# Autodesk Inventor assembly: Ensamble
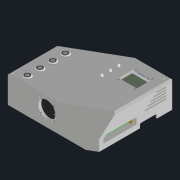
[picture p0: Inventor's stored thumbnail of the model, 180x180]
Saved by Autodesk Inventor 2022 (Build 260153000, 153)
## iProperties
Created: 2022-01-04
Part Number: Ensamble
Document SubType Name: Assembly
Designer: Andres
Author: Andres
## Documents named in this file (22)
- D:\Documentos\Proyectos Personales\SistemaSeguridad\cad\Ensamble.iam
- D:\Documentos\Proyectos Personales\SistemaSeguridad\cad\base.ipt
- D:\Documentos\Proyectos Personales\SistemaSeguridad\cad\mainboard.ipt
- D:\Documentos\Proyectos Personales\SistemaSeguridad\cad\Ardi_UNO.ipt
- D:\Documentos\Proyectos Personales\SistemaSeguridad\cad\4_Relay_module_Simplify_1.ipt
- D:\Documentos\Proyectos Personales\SistemaSeguridad\cad\nokia-5110-lcd-graphic-84x48-pixel-arduiono-compatible-blue-board-1.snapshot.2\Nokia LCD.ipt
- D:\Documentos\Proyectos Personales\SistemaSeguridad\cad\AC-DC transformer.ipt
- D:\Documentos\Proyectos Personales\SistemaSeguridad\cad\Cubierta.ipt
- D:\Documentos\Inventor\Content Center Files\R2022\en-US\ISO 4762(2)\ISO 4762 - M3 x 30ISO.ipt
- D:\Documentos\Inventor\Content Center Files\R2022\en-US\ISO 4032(2)\ISO 4032 - M3 - ISO.ipt
- D:\Documentos\Inventor\Content Center Files\R2022\en-US\ISO 4762(2)\ISO 4762 - M3 x 8ISO.ipt
- D:\Documentos\Proyectos Personales\SistemaSeguridad\cad\led-push-button-1.snapshot.1\LED-BUTTON.ipt
- D:\Documentos\Proyectos Personales\SistemaSeguridad\cad\speaker.ipt
- D:\Documentos\Proyectos Personales\SistemaSeguridad\cad\40x40x10mm-brushless-axial-fan-1.snapshot.2\model.ipt
- fan.ipt
- D:\Documentos\Proyectos Personales\SistemaSeguridad\cad\led-5mm-1.snapshot.6\LED 5mm.ipt
- D:\Documentos\Proyectos Personales\SistemaSeguridad\cad\spacer-m3-l5-l70-1.snapshot.2\Spacer Bolts_m3_bn_L6.ipt
- D:\Documentos\Inventor\Content Center Files\R2022\en-US\ISO 7045  Z\ISO 7045 - M2.5 x 4_ - 4.8 - Z - ISO.ipt
- D:\Documentos\Inventor\Content Center Files\R2022\en-US\ISO 7045  Z\ISO 7045 - M3 x 5_ - 4.8 - Z - ISO.ipt
- D:\Documentos\Inventor\Content Center Files\R2022\en-US\ISO 7045  Z\ISO 7045 - M2.5 x 5_ - 4.8 - Z - ISO.ipt
- D:\Documentos\Inventor\Content Center Files\R2022\en-US\ISO 4762(2)\ISO 4762 - M3 x 12ISO.ipt
- D:\Documentos\Inventor\Content Center Files\R2022\en-US\ISO 4762(2)\ISO 4762 - M3 x 16ISO.ipt
## Components (79 placed, 20 different names)
1. base:1 — Mate:1, Mate:2, Mate:3, Flush:5, Flush:6, Flush:7, Flush:8, Flush:9, Mate:5, Flush:10, Mate:13, Mate:15, Mate:41, Mate:42, Angle:1, Mate:72, Mate:73, Mate:74, Mate:75, Mate:76, Mate:77, Mate:78, Mate:79, Mate:80, Mate:81, Mate:82, Mate:83, Mate:84, Mate:85, Mate:86, Mate:87, Mate:88, Mate:89, Mate:90, Mate:91, Mate:92, Mate:93, Mate:94, Mate:95, Mate:104
2. mainboard:1 — Mate:1, Flush:6, Mate:4, Mate:40, Flush:11, Mate:96, Mate:97, Mate:98, Mate:99, Mate:100, Mate:101, Mate:102, Mate:103, Mate:105
3. Ardi_UNO:1 — Mate:2, Flush:5, Flush:8, Mate:4, Insert:5, Insert:6, Insert:7, Insert:8
4. 4_Relay_module_Simplify_1:1 — Mate:3, Flush:7, Flush:9, Insert:1, Insert:2, Insert:3, Insert:4
5. Nokia LCD:1 — Mate:6, Mate:7, Mate:25, Mate:27, Mate:29, Mate:31
6. AC-DC transformer:1 — Mate:5, Mate:40, Flush:11
7. Cubierta:1 — Flush:10, Mate:6, Mate:7, Mate:8, Mate:9, Mate:10, Mate:11, Mate:12, Mate:14, Mate:16, Mate:17, Mate:18, Mate:19, Mate:20, Mate:21, Mate:22, Mate:23, Mate:24, Mate:26, Mate:28, Mate:30, Mate:32, Mate:33, Mate:34, Mate:35, Mate:36, Mate:37, Mate:38, Mate:39, Mate:43, Mate:44, Mate:45, Mate:46, Mate:47, Mate:48, Mate:49, Mate:50, Mate:51, Mate:52, Mate:53, Mate:54, Mate:56, Mate:58, Mate:60, Mate:66, Mate:67, Mate:68, Mate:69, Mate:70, Mate:71
8. ISO 4762 M3 x 30:1 — Mate:8, Mate:9
9. ISO 4032 M3:1 — Mate:12, Mate:13
10. ISO 4762 M3 x 30:2 — Mate:10, Mate:11
11. ISO 4032 M3:2 — Mate:14, Mate:15
12. ISO 4762 M3 x 8:1 — Mate:16, Mate:17
13. ISO 4032 M3:3 — Mate:24, Mate:25
14. ISO 4762 M3 x 8:2 — Mate:18, Mate:19
15. ISO 4762 M3 x 8:3 — Mate:20, Mate:21
16. ISO 4762 M3 x 8:4 — Mate:22, Mate:23
17. ISO 4032 M3:4 — Mate:26, Mate:27
18. ISO 4032 M3:5 — Mate:28, Mate:29
19. ISO 4032 M3:6 — Mate:30, Mate:31
20. LED-BUTTON:1 — Mate:32, Mate:33
21. LED-BUTTON:2 — Mate:34, Mate:39
22. LED-BUTTON:3 — Mate:36, Mate:37
23. LED-BUTTON:4 — Mate:35, Mate:38
24. speaker:1 — Mate:41, Mate:42, Angle:1, Insert:25, Insert:26
25. fan:1 — Mate:43, Mate:44, Mate:45, Mate:55, Mate:57, Mate:59, Mate:61
26. ISO 4762 M3 x 16:1 — Mate:46, Mate:47
27. ISO 4032 M3:7 — Mate:54, Mate:55
28. ISO 4762 M3 x 16:2 — Mate:48, Mate:49
29. ISO 4762 M3 x 16:3 — Mate:50, Mate:51
30. ISO 4762 M3 x 16:4 — Mate:52, Mate:53
31. ISO 4032 M3:8 — Mate:56, Mate:57
32. ISO 4032 M3:9 — Mate:58, Mate:59
33. ISO 4032 M3:10 — Mate:60, Mate:61
34. LED 5mm:3 — Mate:66, Mate:67
35. LED 5mm:4 — Mate:68, Mate:71
36. LED 5mm:5 — Mate:69, Mate:70
37. Spacer Bolts_m3_bn_L6:1 — Mate:76, Mate:79
38. Spacer Bolts_m3_bn_L6:2 — Mate:75, Mate:78
39. Spacer Bolts_m3_bn_L6:3 — Mate:72, Mate:73
40. Spacer Bolts_m3_bn_L6:4 — Mate:74, Mate:77
41. Spacer Bolts_m3_bn_L6:5 — Mate:80, Mate:84
42. Spacer Bolts_m3_bn_L6:6 — Mate:81, Mate:87
43. Spacer Bolts_m3_bn_L6:7 — Mate:83, Mate:85
44. Spacer Bolts_m3_bn_L6:8 — Mate:82, Mate:86
45. Spacer Bolts_m3_bn_L6:9 — Mate:91, Mate:94
46. Spacer Bolts_m3_bn_L6:10 — Mate:90, Mate:95
47. Spacer Bolts_m3_bn_L6:11 — Mate:89, Mate:92
48. Spacer Bolts_m3_bn_L6:12 — Mate:88, Mate:93
49. ISO 7045 Z M2.5 x 5 - 4.8 - Z:1 — Insert:1
50. ISO 7045 Z M2.5 x 4 - 4.8 - Z:2 — Insert:2
51. ISO 7045 Z M2.5 x 4 - 4.8 - Z:3 — Insert:3
52. ISO 7045 Z M2.5 x 4 - 4.8 - Z:4 — Insert:4
53. ISO 7045 Z M3 x 5 - 4.8 - Z:5 — Insert:5
54. ISO 7045 Z M3 x 5 - 4.8 - Z:6 — Insert:6
55. ISO 7045 Z M3 x 5 - 4.8 - Z:7 — Insert:7
56. ISO 7045 Z M3 x 5 - 4.8 - Z:8 — Insert:8
57. ISO 7045 Z M3 x 5 - 4.8 - Z:9 — Mate:96, Mate:97
58. ISO 7045 Z M3 x 5 - 4.8 - Z:1 — Mate:98, Mate:99
59. ISO 7045 Z M3 x 5 - 4.8 - Z:2 — Mate:100, Mate:101
60. ISO 7045 Z M3 x 5 - 4.8 - Z:3 — Mate:102, Mate:103
61. ISO 7045 Z M3 x 5 - 4.8 - Z:4 — Mate:104, Mate:105
62. ISO 4032 M3:11
63. ISO 4032 M3:12
64. ISO 4032 M3:13
65. ISO 4032 M3:14
66. ISO 4032 M3:15
67. ISO 4032 M3:16
68. ISO 4032 M3:17
69. ISO 4032 M3:18
70. ISO 4032 M3:19
71. ISO 4032 M3:20
72. ISO 4032 M3:21
73. ISO 4032 M3:22
74. ISO 4032 M3:23
75. ISO 4032 M3:24
76. ISO 4032 M3:25
77. ISO 4032 M3:26
78. ISO 4762 M3 x 12:1 — Insert:25
79. ISO 4762 M3 x 12:2 — Insert:26
## Relationships (135: Mate 101, Insert 26, Flush 7, Angle 1)
- Mate:1 (6 mm): base:1 ↔ mainboard:1
- Mate:2 (6 mm): base:1 ↔ Ardi_UNO:1
- Mate:3 (6 mm): base:1 ↔ 4_Relay_module_Simplify_1:1
- Flush:5 (16 mm): base:1 ↔ Ardi_UNO:1
- Flush:6 (10 mm): base:1 ↔ mainboard:1
- Flush:7 (25 mm): base:1 ↔ 4_Relay_module_Simplify_1:1
- Flush:8 (10 mm): base:1 ↔ Ardi_UNO:1
- Flush:9 (8 mm): base:1 ↔ 4_Relay_module_Simplify_1:1
- Mate:4 (3 mm): mainboard:1 ↔ Ardi_UNO:1
- Mate:5: base:1 ↔ AC-DC transformer:1
- Flush:10: base:1 ↔ Cubierta:1
- Mate:6: Nokia LCD:1 ↔ Cubierta:1
- Mate:7: Nokia LCD:1 ↔ Cubierta:1
- Mate:8: Cubierta:1 ↔ ISO 4762 M3 x 30:1
- Mate:9: Cubierta:1 ↔ ISO 4762 M3 x 30:1
- Mate:10: Cubierta:1 ↔ ISO 4762 M3 x 30:2
- Mate:11: Cubierta:1 ↔ ISO 4762 M3 x 30:2
- Mate:12: Cubierta:1 ↔ ISO 4032 M3:1
- Mate:13: base:1 ↔ ISO 4032 M3:1
- Mate:14: Cubierta:1 ↔ ISO 4032 M3:2
- Mate:15: base:1 ↔ ISO 4032 M3:2
- Mate:16: Cubierta:1 ↔ ISO 4762 M3 x 8:1
- Mate:17: Cubierta:1 ↔ ISO 4762 M3 x 8:1
- Mate:18: Cubierta:1 ↔ ISO 4762 M3 x 8:2
- Mate:19: Cubierta:1 ↔ ISO 4762 M3 x 8:2
- Mate:20: Cubierta:1 ↔ ISO 4762 M3 x 8:3
- Mate:21: Cubierta:1 ↔ ISO 4762 M3 x 8:3
- Mate:22: Cubierta:1 ↔ ISO 4762 M3 x 8:4
- Mate:23: Cubierta:1 ↔ ISO 4762 M3 x 8:4
- Mate:24: Cubierta:1 ↔ ISO 4032 M3:3
- Mate:25: Nokia LCD:1 ↔ ISO 4032 M3:3
- Mate:26: Cubierta:1 ↔ ISO 4032 M3:4
- Mate:27: Nokia LCD:1 ↔ ISO 4032 M3:4
- Mate:28: Cubierta:1 ↔ ISO 4032 M3:5
- Mate:29: Nokia LCD:1 ↔ ISO 4032 M3:5
- Mate:30: Cubierta:1 ↔ ISO 4032 M3:6
- Mate:31: Nokia LCD:1 ↔ ISO 4032 M3:6
- Mate:32: Cubierta:1 ↔ LED-BUTTON:1
- Mate:33: Cubierta:1 ↔ LED-BUTTON:1
- Mate:34: Cubierta:1 ↔ LED-BUTTON:2
- Mate:35: Cubierta:1 ↔ LED-BUTTON:4
- Mate:36: Cubierta:1 ↔ LED-BUTTON:3
- Mate:37: Cubierta:1 ↔ LED-BUTTON:3
- Mate:38: Cubierta:1 ↔ LED-BUTTON:4
- Mate:39: Cubierta:1 ↔ LED-BUTTON:2
- Mate:40 (20 mm): mainboard:1 ↔ AC-DC transformer:1
- Flush:11: mainboard:1 ↔ AC-DC transformer:1
- Mate:41: base:1 ↔ speaker:1
- Mate:42: base:1 ↔ speaker:1
- Angle:1 (45 deg): base:1 ↔ speaker:1
- Mate:43: Cubierta:1 ↔ fan:1
- Mate:44: Cubierta:1 ↔ fan:1
- Mate:45: Cubierta:1 ↔ fan:1
- Mate:46: Cubierta:1 ↔ ISO 4762 M3 x 16:1
- Mate:47: Cubierta:1 ↔ ISO 4762 M3 x 16:1
- Mate:48: Cubierta:1 ↔ ISO 4762 M3 x 16:2
- Mate:49: Cubierta:1 ↔ ISO 4762 M3 x 16:2
- Mate:50: Cubierta:1 ↔ ISO 4762 M3 x 16:3
- Mate:51: Cubierta:1 ↔ ISO 4762 M3 x 16:3
- Mate:52: Cubierta:1 ↔ ISO 4762 M3 x 16:4
- Mate:53: Cubierta:1 ↔ ISO 4762 M3 x 16:4
- Mate:54: Cubierta:1 ↔ ISO 4032 M3:7
- Mate:55: fan:1 ↔ ISO 4032 M3:7
- Mate:56: Cubierta:1 ↔ ISO 4032 M3:8
- Mate:57: fan:1 ↔ ISO 4032 M3:8
- Mate:58: Cubierta:1 ↔ ISO 4032 M3:9
- Mate:59: fan:1 ↔ ISO 4032 M3:9
- Mate:60: Cubierta:1 ↔ ISO 4032 M3:10
- Mate:61: fan:1 ↔ ISO 4032 M3:10
- Mate:66: Cubierta:1 ↔ LED 5mm:3
- Mate:67: Cubierta:1 ↔ LED 5mm:3
- Mate:68: Cubierta:1 ↔ LED 5mm:4
- Mate:69: Cubierta:1 ↔ LED 5mm:5
- Mate:70: Cubierta:1 ↔ LED 5mm:5
- Mate:71: Cubierta:1 ↔ LED 5mm:4
- Mate:72: base:1 ↔ Spacer Bolts_m3_bn_L6:3
- Mate:73: base:1 ↔ Spacer Bolts_m3_bn_L6:3
- Mate:74: base:1 ↔ Spacer Bolts_m3_bn_L6:4
- Mate:75: base:1 ↔ Spacer Bolts_m3_bn_L6:2
- Mate:76: base:1 ↔ Spacer Bolts_m3_bn_L6:1
- Mate:77: base:1 ↔ Spacer Bolts_m3_bn_L6:4
- Mate:78: base:1 ↔ Spacer Bolts_m3_bn_L6:2
- Mate:79: base:1 ↔ Spacer Bolts_m3_bn_L6:1
- Mate:80: base:1 ↔ Spacer Bolts_m3_bn_L6:5
- Mate:81: base:1 ↔ Spacer Bolts_m3_bn_L6:6
- Mate:82: base:1 ↔ Spacer Bolts_m3_bn_L6:8
- Mate:83: base:1 ↔ Spacer Bolts_m3_bn_L6:7
- Mate:84: base:1 ↔ Spacer Bolts_m3_bn_L6:5
- Mate:85: base:1 ↔ Spacer Bolts_m3_bn_L6:7
- Mate:86: base:1 ↔ Spacer Bolts_m3_bn_L6:8
- Mate:87: base:1 ↔ Spacer Bolts_m3_bn_L6:6
- Mate:88: base:1 ↔ Spacer Bolts_m3_bn_L6:12
- Mate:89: base:1 ↔ Spacer Bolts_m3_bn_L6:11
- Mate:90: base:1 ↔ Spacer Bolts_m3_bn_L6:10
- Mate:91: base:1 ↔ Spacer Bolts_m3_bn_L6:9
- Mate:92: base:1 ↔ Spacer Bolts_m3_bn_L6:11
- Mate:93: base:1 ↔ Spacer Bolts_m3_bn_L6:12
- Mate:94: base:1 ↔ Spacer Bolts_m3_bn_L6:9
- Mate:95: base:1 ↔ Spacer Bolts_m3_bn_L6:10
- Insert:1: 4_Relay_module_Simplify_1:1 ↔ ISO 7045 Z M2.5 x 5 - 4.8 - Z:1
- Insert:2: 4_Relay_module_Simplify_1:1 ↔ ISO 7045 Z M2.5 x 4 - 4.8 - Z:2
- Insert:3: 4_Relay_module_Simplify_1:1 ↔ ISO 7045 Z M2.5 x 4 - 4.8 - Z:3
- Insert:4: 4_Relay_module_Simplify_1:1 ↔ ISO 7045 Z M2.5 x 4 - 4.8 - Z:4
- Insert:5: Ardi_UNO:1 ↔ ISO 7045 Z M3 x 5 - 4.8 - Z:5
- Insert:6: Ardi_UNO:1 ↔ ISO 7045 Z M3 x 5 - 4.8 - Z:6
- Insert:7: Ardi_UNO:1 ↔ ISO 7045 Z M3 x 5 - 4.8 - Z:7
- Insert:8: Ardi_UNO:1 ↔ ISO 7045 Z M3 x 5 - 4.8 - Z:8
- Mate:96: mainboard:1 ↔ ISO 7045 Z M3 x 5 - 4.8 - Z:9
- Mate:97: mainboard:1 ↔ ISO 7045 Z M3 x 5 - 4.8 - Z:9
- Mate:98: mainboard:1 ↔ ISO 7045 Z M3 x 5 - 4.8 - Z:1
- Mate:99: mainboard:1 ↔ ISO 7045 Z M3 x 5 - 4.8 - Z:1
- Mate:100: mainboard:1 ↔ ISO 7045 Z M3 x 5 - 4.8 - Z:2
- Mate:101: mainboard:1 ↔ ISO 7045 Z M3 x 5 - 4.8 - Z:2
- Mate:102: mainboard:1 ↔ ISO 7045 Z M3 x 5 - 4.8 - Z:3
- Mate:103: mainboard:1 ↔ ISO 7045 Z M3 x 5 - 4.8 - Z:3
- Mate:104: base:1 ↔ ISO 7045 Z M3 x 5 - 4.8 - Z:4
- Mate:105: mainboard:1 ↔ ISO 7045 Z M3 x 5 - 4.8 - Z:4
- [Insert]: base:1 ↔ ISO 4032 M3:11
- [Insert]: base:1 ↔ ISO 4032 M3:12
- [Insert]: base:1 ↔ ISO 4032 M3:13
- [Insert]: base:1 ↔ ISO 4032 M3:14
- [Insert]: base:1 ↔ ISO 4032 M3:15
- [Insert]: base:1 ↔ ISO 4032 M3:16
- [Insert]: base:1 ↔ ISO 4032 M3:17
- [Insert]: base:1 ↔ ISO 4032 M3:18
- [Insert]: base:1 ↔ ISO 4032 M3:19
- [Insert]: base:1 ↔ ISO 4032 M3:20
- [Insert]: base:1 ↔ ISO 4032 M3:21
- [Insert]: base:1 ↔ ISO 4032 M3:22
- [Insert]: base:1 ↔ ISO 4032 M3:23
- [Insert]: base:1 ↔ ISO 4032 M3:24
- [Insert]: base:1 ↔ ISO 4032 M3:25
- [Insert]: base:1 ↔ ISO 4032 M3:26
- Insert:25: speaker:1 ↔ ISO 4762 M3 x 12:1
- Insert:26: speaker:1 ↔ ISO 4762 M3 x 12:2
